# Autodesk Inventor assembly: Assembled board
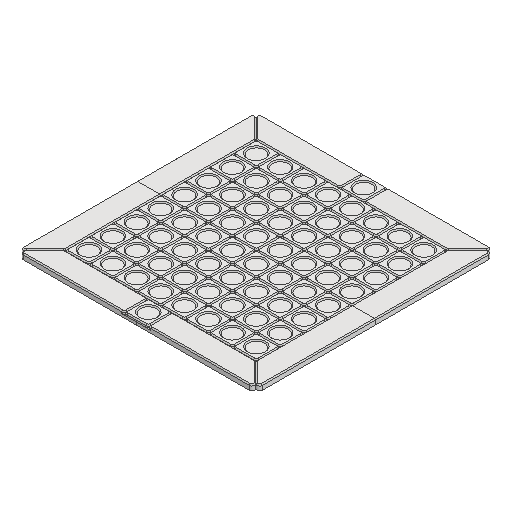
[picture p0: Inventor's stored thumbnail of the model, 512x512]
Saved by Autodesk Inventor 2025.2 (Build 292293000, 293)
## iProperties
Created: 2025-03-03
Part Number: Assembled board
Document SubType Name: Assembly
Designer: Marcu
Author: Marcu
## Documents named in this file (7)
- C:\Users\Marcu\Documents\GitHub\Semesterprojekt-2025\3D filer\Board\Assembled board.iam
- C:\Users\Marcu\Documents\GitHub\Semesterprojekt-2025\3D filer\Board\Base.ipt
- C:\Users\Marcu\Documents\GitHub\Semesterprojekt-2025\3D filer\Board\Top.ipt
- C:\Users\Marcu\Documents\GitHub\Semesterprojekt-2025\3D filer\Board\Border P L.ipt
- C:\Users\Marcu\Documents\GitHub\Semesterprojekt-2025\3D filer\Board\Border P R.ipt
- C:\Users\Marcu\Documents\GitHub\Semesterprojekt-2025\3D filer\Board\Border S 2.ipt
- C:\Users\Marcu\Documents\GitHub\Semesterprojekt-2025\3D filer\Board\Border S 1.ipt
## Components (138 placed, 6 different names)
1. Border P L:1 — Flush:1, Flush:2, Flush:3, Mate:2, Mate:3, Mate:9
2. Border P R:1 — Flush:2, Flush:3, Mate:2, Flush:5, Mate:12
3. Top:65 — Mate:3
4. Border P L:2 — Mate:4, Flush:4, Flush:5, Mate:5, Flush:6, Flush:7, Mate:6, Mate:11
5. Border P R:2 — Mate:5, Flush:6, Flush:7, Mate:10
6. Top:66 — Mate:6
7. Border S 2:1 — Flush:10, Flush:11, Mate:8, Mate:9
8. Border S 2:2 — Mate:7, Flush:8, Flush:9, Mate:11
9. Border S 1:1 — Mate:7, Flush:8, Flush:9, Mate:12
10. Border S 1:2 — Flush:10, Flush:11, Mate:8, Mate:10
11. Base:1 — Mate:1
12. Base:2
13. Base:3
14. Base:4
15. Base:5
16. Base:6
17. Base:7
18. Base:8
19. Base:9
20. Base:10
21. Base:11
22. Base:12
23. Base:13
24. Base:14
25. Base:15
26. Base:16
27. Base:17
28. Base:18
29. Base:19
30. Base:20
31. Base:21
32. Base:22
33. Base:23
34. Base:24
35. Base:25
36. Base:26
37. Base:27
38. Base:28
39. Base:29
40. Base:30
41. Base:31
42. Base:32
43. Base:33
44. Base:34
45. Base:35
46. Base:36
47. Base:37
48. Base:38
49. Base:39
50. Base:40
51. Base:41
52. Base:42
53. Base:43
54. Base:44
55. Base:45
56. Base:46
57. Base:47
58. Base:48
59. Base:49
60. Base:50
61. Base:51
62. Base:52
63. Base:53
64. Base:54
65. Base:55
66. Base:56
67. Base:57
68. Base:58
69. Base:59
70. Base:60
71. Base:61
72. Base:62
73. Base:63
74. Base:64 — Mate:4
75. Top:1 — Mate:1, Flush:4
76. Top:2
77. Top:3
78. Top:4
79. Top:5
80. Top:6
81. Top:7
82. Top:8
83. Top:9
84. Top:10
85. Top:11
86. Top:12
87. Top:13
88. Top:14
89. Top:15
90. Top:16
91. Top:17 — Flush:1
92. Top:18
93. Top:19
94. Top:20
95. Top:21
96. Top:22
97. Top:23
98. Top:24
99. Top:25
100. Top:26
101. Top:27
102. Top:28
103. Top:29
104. Top:30
105. Top:31
106. Top:32
107. Top:33
108. Top:34
109. Top:35
110. Top:36
111. Top:37
112. Top:38
113. Top:39
114. Top:40
115. Top:41
116. Top:42
117. Top:43
118. Top:44
119. Top:45
120. Top:46
121. Top:47
122. Top:48
123. Top:49
124. Top:50
125. Top:51
126. Top:52
127. Top:53
128. Top:54
129. Top:55
130. Top:56
131. Top:57
132. Top:58
133. Top:59
134. Top:60
135. Top:61
136. Top:62
137. Top:63
138. Top:64
## Component patterns: (64 elements, first: Base:1), (64 elements, first: Top:1)
## Relationships (23: Mate 12, Flush 11)
- Mate:1: Base:1 ↔ Top:1
- Flush:1: Border P L:1 ↔ Top:17
- Flush:2: Border P L:1 ↔ Border P R:1
- Flush:3: Border P L:1 ↔ Border P R:1
- Mate:2: Border P L:1 ↔ Border P R:1
- Mate:3: Border P L:1 ↔ Top:65
- Mate:4: Border P L:2 ↔ Base:64
- Flush:4: Border P L:2 ↔ Top:1
- Flush:5: Border P R:1 ↔ Border P L:2
- Mate:5: Border P L:2 ↔ Border P R:2
- Flush:6: Border P L:2 ↔ Border P R:2
- Flush:7: Border P L:2 ↔ Border P R:2
- Mate:6: Border P L:2 ↔ Top:66
- Mate:7: Border S 2:2 ↔ Border S 1:1
- Flush:8: Border S 2:2 ↔ Border S 1:1
- Flush:9: Border S 2:2 ↔ Border S 1:1
- Flush:10: Border S 2:1 ↔ Border S 1:2
- Flush:11: Border S 2:1 ↔ Border S 1:2
- Mate:8: Border S 2:1 ↔ Border S 1:2
- Mate:9: Border P L:1 ↔ Border S 2:1
- Mate:10: Border P R:2 ↔ Border S 1:2
- Mate:11: Border P L:2 ↔ Border S 2:2
- Mate:12: Border P R:1 ↔ Border S 1:1
